# Autodesk Inventor assembly: Differential Swerve Drive V1
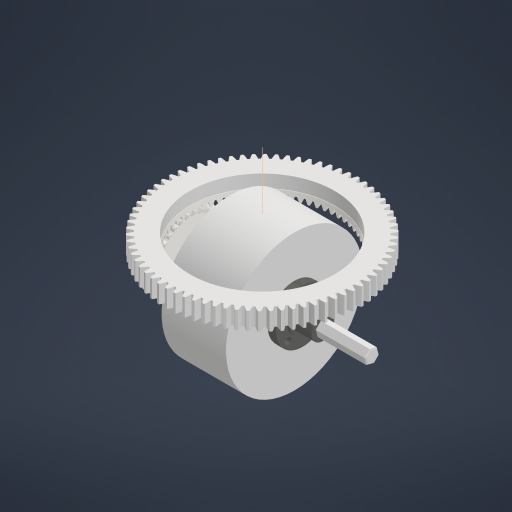
[picture p0: Inventor's stored thumbnail of the model, 512x512]
Saved by Autodesk Inventor 2023 (Build 270158000, 158)
## iProperties
Created: 2023-08-02
Part Number: Differential Swerve Drive V1
Document SubType Name: Assembly
Designer: izack
Author: izack
## Documents named in this file (9)
- F:\CAD Modeling\Private Robotics\Custom Tryhard Robot\Drivetrain\Custom-Modules-CAD\Differential Swerve Drive V1\Differential Swerve Drive V1.iam
- F:\CAD Modeling\Private Robotics\Custom Tryhard Robot\Drivetrain\Custom-Modules-CAD\Differential Swerve Drive V1\60mm_Grip_Wheel.ipt
- F:\CAD Modeling\Private Robotics\Custom Tryhard Robot\Drivetrain\Custom-Modules-CAD\Differential Swerve Drive V1\Differential Swerve Drive Parts\High Strength Hub.ipt
- C:\Users\Izack Waczko\Documents\Ring Gear Base.ipt
- F:\CAD Modeling\Private Robotics\Custom Tryhard Robot\Drivetrain\Custom-Modules-CAD\FalseAxle.ipt
- F:\CAD Modeling\Private Robotics\Custom Tryhard Robot\Drivetrain\Custom-Modules-CAD\Differential Swerve Drive V1\Differential Swerve Drive Parts\5mm x 55mm Hex Shaft.ipt
- F:\CAD Modeling\Private Robotics\Custom Tryhard Robot\Drivetrain\Custom-Modules-CAD\False Axle.ipt
- F:\CAD Modeling\Private Robotics\Custom Tryhard Robot\Drivetrain\Custom-Modules-CAD\Differential Swerve Drive V1\Differential Swerve Drive V1\Design Accelerator\Bevel Gears1.iam
- F:\CAD Modeling\Private Robotics\Custom Tryhard Robot\Drivetrain\Custom-Modules-CAD\Differential Swerve Drive V1\Differential Swerve Drive V1\Design Accelerator\Bevel Gears2.iam
## Components (9 placed, 7 different names)
1. 60mm_Grip_Wheel:1 — Mate:1, Mate:2, Mate:3, Mate:4, Mate:5, Mate:6
2. High Strength Hub:1 — Mate:4, Mate:5, Mate:6
3. High Strength Hub:2 — Mate:1, Mate:2, Mate:3, Mate:7, Mate:8
4. Ring Gear Base:1 — Flush:1, Mate:9, Angle:1, Flush:4
5. FalseAxle:1 — Flush:2
6. 5mm x 55mm Hex Shaft:1 — Mate:7, Mate:8, Flush:3
7. False Axle:1 — Flush:3, Mate:10, Angle:2
8. Bevel Gears:1 [sub-assembly] — Mate:9, Angle:1, Flush:4
9. Bevel Gears:2 [sub-assembly] — Mate:10, Angle:2
## Relationships (16: Mate 10, Flush 4, Angle 2)
- Mate:1: 60mm_Grip_Wheel:1 ↔ High Strength Hub:2
- Mate:2: 60mm_Grip_Wheel:1 ↔ High Strength Hub:2
- Mate:3: 60mm_Grip_Wheel:1 ↔ High Strength Hub:2
- Mate:4: 60mm_Grip_Wheel:1 ↔ High Strength Hub:1
- Mate:5: 60mm_Grip_Wheel:1 ↔ High Strength Hub:1
- Mate:6: 60mm_Grip_Wheel:1 ↔ High Strength Hub:1
- Flush:1 (11.5 mm): Ring Gear Base:1
- Flush:2: FalseAxle:1
- Mate:7: High Strength Hub:2 ↔ 5mm x 55mm Hex Shaft:1
- Mate:8: High Strength Hub:2 ↔ 5mm x 55mm Hex Shaft:1
- Flush:3: 5mm x 55mm Hex Shaft:1 ↔ False Axle:1
- Mate:9: Ring Gear Base:1 ↔ Bevel Gears:1
- Angle:1 (0 deg): Ring Gear Base:1 ↔ Bevel Gears:1
- Flush:4: Ring Gear Base:1 ↔ Bevel Gears:1
- Mate:10: False Axle:1 ↔ Bevel Gears:2
- Angle:2 (0 deg): False Axle:1 ↔ Bevel Gears:2
